# Autodesk Inventor assembly: Room_Full
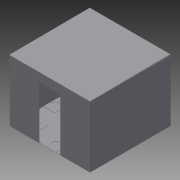
[picture p0: Inventor's stored thumbnail of the model, 180x180]
Saved by Autodesk Inventor 2013 (Build 170138000, 138)
## iProperties
Created: 2011-06-21
Part Number: Room_Full
Document SubType Name: Assembly
Designer: rrw
Author: rrw
## Documents named in this file (5)
- C:\Users\JCH4\Documents\Steckler_Compartment\Updated_Files\Room_Full(updated).iam
- C:\Users\JCH4\Documents\Steckler_Compartment\Wall_door.ipt
- C:\Users\JCH4\Documents\Steckler_Compartment\floor.ipt
- C:\Users\JCH4\Documents\Steckler_Compartment\Wall_back.ipt
- C:\Users\JCH4\Documents\Steckler_Compartment\fire_locs.ipt
## Components (7 placed, 4 different names)
1. Wall_door:1 — Mate:1, Mate:2, Mate:6, Mate:8, Mate:12
2. floor:1 — Mate:1, Mate:2, Mate:3, Mate:4, Mate:7, Mate:11, Flush:1
3. Wall_back:1 — Mate:3, Mate:4, Mate:5, Mate:9, Mate:10
4. Wall_back:2 — Mate:5, Mate:6, Mate:7, Mate:8, Mate:9, Mate:13, Mate:14
5. Wall_back:3 — Mate:10, Mate:11
6. floor:2 — Mate:12, Mate:13, Mate:14
7. fire_locs:1 — Flush:1
## Relationships (15: Mate 14, Flush 1)
- Mate:1: Wall_door:1 ↔ floor:1
- Mate:2: Wall_door:1 ↔ floor:1
- Mate:3: floor:1 ↔ Wall_back:1
- Mate:4: floor:1 ↔ Wall_back:1
- Mate:5: Wall_back:1 ↔ Wall_back:2
- Mate:6: Wall_door:1 ↔ Wall_back:2
- Mate:7: floor:1 ↔ Wall_back:2
- Mate:8: Wall_door:1 ↔ Wall_back:2
- Mate:9: Wall_back:1 ↔ Wall_back:2
- Mate:10: Wall_back:1 ↔ Wall_back:3
- Mate:11: floor:1 ↔ Wall_back:3
- Mate:12: Wall_door:1 ↔ floor:2
- Mate:13: Wall_back:2 ↔ floor:2
- Mate:14: Wall_back:2 ↔ floor:2
- Flush:1: floor:1 ↔ fire_locs:1
